# Autodesk Inventor assembly: Assembly1
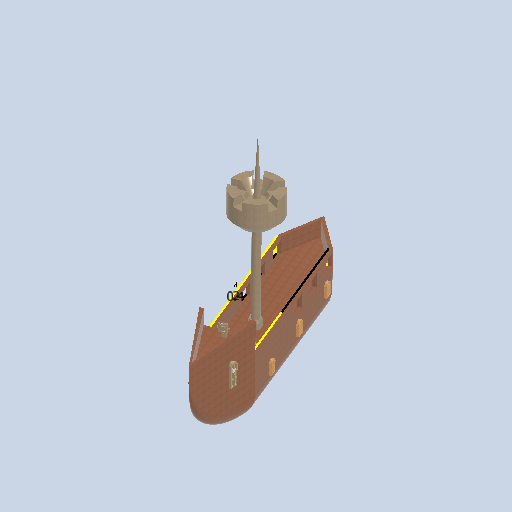
[picture p0: Inventor's stored thumbnail of the model, 512x512]
Saved by Autodesk Inventor 2024.1 (Build 281209000, 209)
## iProperties
Created: 2023-11-09
Part Number: Assembly1
Document SubType Name: Assembly
Designer: luvag
Author: luvag
## Documents named in this file (3)
- C:\Users\luvag\Desktop\Assembly1.iam
- C:\Users\luvag\Desktop\Assembly6.iam
- C:\Users\luvag\Desktop\Maitri_table.ipt
## Components (2 placed, 2 different names)
1. Assembly6:1 [sub-assembly]
2. Maitri_table:1
## Relationships (1: Mate 1)
- [Mate]: Assembly6:1 ↔ Maitri_table:1
